# Autodesk Inventor assembly: DribblerUnit
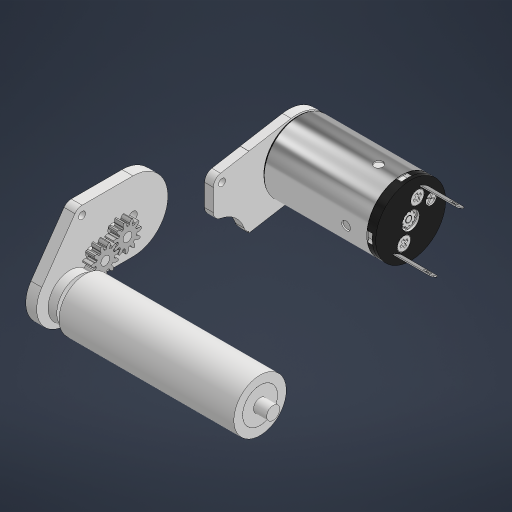
[picture p0: Inventor's stored thumbnail of the model, 512x512]
Saved by Autodesk Inventor 2024.2 (Build 282272000, 272)
## iProperties
Created: 2023-12-27
Part Number: DribblerUnit
Document SubType Name: Assembly
Designer: Hanaoka
Author: Hanaoka
## Documents named in this file (13)
- G:\共有ドライブ\reRo\05_個人\hanaoka\inventor\DribblerUnit\DribblerUnit.iam
- G:\共有ドライブ\reRo\05_個人\hanaoka\inventor\DribblerUnit\Dribbler_Tube.ipt
- G:\共有ドライブ\reRo\05_個人\hanaoka\inventor\DribblerUnit\Shaft_350.ipt
- G:\共有ドライブ\reRo\05_個人\hanaoka\inventor\DribblerUnit\Bearing_C-FL673ZZ\Bearing_C-FL673ZZ.ipt
- G:\共有ドライブ\reRo\05_個人\hanaoka\inventor\DribblerUnit\Tube_Hub.ipt
- G:\共有ドライブ\reRo\05_個人\hanaoka\inventor\DribblerUnit\Althonix16dct\Althonix16dct.ipt
- G:\共有ドライブ\reRo\05_個人\hanaoka\inventor\HandleUnit\MotorMount.ipt
- G:\共有ドライブ\reRo\05_個人\hanaoka\inventor\HandleUnit\GearCover.ipt
- G:\共有ドライブ\reRo\05_個人\hanaoka\inventor\HandleUnit\OutSide_Gear.ipt
- G:\共有ドライブ\reRo\05_個人\hanaoka\inventor\DribblerUnit\Gear_M0.5_8T_D4\Gear_M0.5_8T_D4.ipt
- G:\共有ドライブ\reRo\05_個人\hanaoka\inventor\Screw\M1.7x5.ipt
- G:\共有ドライブ\reRo\05_個人\hanaoka\inventor\Screw\Shaft_2x6.ipt
- G:\共有ドライブ\reRo\05_個人\hanaoka\inventor\DribblerUnit\Gear_M0.5_11T_D5.5\Gear_M0.5_11T_D5.5.ipt
## Components (16 placed, 12 different names)
1. Dribbler_Tube:1 — 挿入:2
2. Shaft_350:1 — 挿入:1, 挿入:4, 挿入:8
3. Bearing_C-FL673ZZ:1 — 挿入:1, 挿入:6
4. Tube_Hub:1 — 挿入:2, 挿入:4
5. Althonix16dct:1 — 挿入:5, メイト:1, 挿入:9
6. MotorMount:1 — 挿入:5, メイト:1, 挿入:10, 挿入:11, 挿入:12
7. GearCover:1 — 挿入:6, 挿入:15, 挿入:16
8. OutSide_Gear:1 — 挿入:8
9. Gear_M0.5_8T_D4:1 — 挿入:9
10. M1.7x5:1 — 挿入:10
11. M1.7x5:2 — 挿入:12
12. M1.7x5:3 — 挿入:11
13. Shaft_2x6:1 — 挿入:14, 挿入:15
14. Gear_M0.5_11T_D5.5:1 — 挿入:14
15. Gear_M0.5_11T_D5.5:2 — 挿入:13
16. Shaft_2x6:2 — 挿入:13, 挿入:16
## Relationships (15: Insert 14, Mate 1)
- 挿入:1 [Insert]: Shaft_350:1 ↔ Bearing_C-FL673ZZ:1
- 挿入:2 [Insert]: Dribbler_Tube:1 ↔ Tube_Hub:1
- 挿入:4 [Insert] (12 mm): Shaft_350:1 ↔ Tube_Hub:1
- 挿入:5 [Insert]: Althonix16dct:1 ↔ MotorMount:1
- メイト:1 [Mate]: Althonix16dct:1 ↔ MotorMount:1
- 挿入:6 [Insert]: Bearing_C-FL673ZZ:1 ↔ GearCover:1
- 挿入:8 [Insert] (3.5 mm): Shaft_350:1 ↔ OutSide_Gear:1
- 挿入:9 [Insert] (2 mm): Althonix16dct:1 ↔ Gear_M0.5_8T_D4:1
- 挿入:10 [Insert]: MotorMount:1 ↔ M1.7x5:1
- 挿入:11 [Insert]: MotorMount:1 ↔ M1.7x5:3
- 挿入:12 [Insert]: MotorMount:1 ↔ M1.7x5:2
- 挿入:13 [Insert]: Gear_M0.5_11T_D5.5:2 ↔ Shaft_2x6:2
- 挿入:14 [Insert]: Shaft_2x6:1 ↔ Gear_M0.5_11T_D5.5:1
- 挿入:15 [Insert]: GearCover:1 ↔ Shaft_2x6:1
- 挿入:16 [Insert]: GearCover:1 ↔ Shaft_2x6:2
